# Autodesk Inventor assembly: Stand
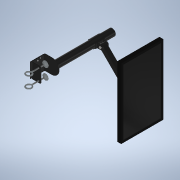
[picture p0: Inventor's stored thumbnail of the model, 180x180]
Saved by Autodesk Inventor 2020 (Build 240168000, 168)
## iProperties
Created: 2021-07-08
Part Number: Stand
Document SubType Name: Assembly
Designer: Simon.Alvarez
Mass: 3004.31 g
Surface Area: 3337 cm^2
Volume: 382.876 cm^3
Density: 7.84669 g/cm^3
Author: Simon.Alvarez
## Documents named in this file (9)
- C:\Users\Simon.Alvarez\Desktop\Simon off laptop\Desk\Monitor Stand\Stand.iam
- C:\Users\Simon.Alvarez\Desktop\Simon off laptop\Desk\Monitor Stand\Pole.ipt
- C:\Users\Simon.Alvarez\Desktop\Simon off laptop\Desk\Monitor Stand\Clamp_Plate.ipt
- C:\Users\Simon.Alvarez\Documents\Inventor\Content Center Files\R2020\en-US\BS EN ISO 7045 Z\EN ISO 7045 - M8 x 10 - 4.8 - Z(1).ipt
- C:\Users\Simon.Alvarez\Desktop\Simon off laptop\Desk\Monitor Stand\Clamp Thread.ipt
- C:\Users\Simon.Alvarez\Documents\Inventor\Content Center Files\R2020\en-US\BS EN ISO 7045 Z\EN ISO 7045 - M6 x 12 - 4.8 - Z(1).ipt
- C:\Users\Simon.Alvarez\Desktop\Simon off laptop\Desk\Monitor Stand\Arm.iam
- C:\Users\Simon.Alvarez\Desktop\Simon off laptop\Desk\Monitor Stand\Monitor_21inch.ipt
- C:\Users\Simon.Alvarez\Documents\Inventor\Content Center Files\R2020\en-US\BS EN ISO 7045 Z\EN ISO 7045 - M4 x 5 - 4.8 - Z(1).ipt
## Components (14 placed, 8 different names)
1. Pole:1 — Flush:1, Flush:2, Flush:3, Mate:1, Mate:2, Mate:3, Insert:1, Insert:2, Mate:7, Mate:8
2. Clamp_Plate:1 — Mate:1, Mate:2, Mate:3, Mate:4, Mate:5
3. BS EN ISO 7045 Z - Metric M8 x 10 - 4.8 - Z:1 — Insert:1
4. BS EN ISO 7045 Z - Metric M8 x 10 - 4.8 - Z:2 — Insert:2
5. Clamp Thread:1 — Mate:4, Mate:6
6. Clamp Thread:2 — Mate:5, Mate:6
7. Arm:1 [sub-assembly] — Mate:7, Mate:8, Mate:9, Tangent:1, Mate:10, Tangent:2, Mate:11, Mate:12, Mate:13, Insert:3, Insert:4, Insert:5, Insert:6
8. BS EN ISO 7045 Z - Metric M6 x 12 - 4.8 - Z:1 — Mate:9, Tangent:1
9. BS EN ISO 7045 Z - Metric M6 x 12 - 4.8 - Z:2 — Mate:10, Tangent:2
10. Monitor_21inch:1 — Mate:11, Mate:12, Mate:13
11. BS EN ISO 7045 Z - Metric M4 x 5 - 4.8 - Z:1 — Insert:3
12. BS EN ISO 7045 Z - Metric M4 x 5 - 4.8 - Z:2 — Insert:4
13. BS EN ISO 7045 Z - Metric M4 x 5 - 4.8 - Z:3 — Insert:5
14. BS EN ISO 7045 Z - Metric M4 x 5 - 4.8 - Z:4 — Insert:6
## Relationships (24: Mate 13, Insert 6, Flush 3, Tangent 2)
- Flush:1: Pole:1
- Flush:2: Pole:1
- Flush:3: Pole:1
- Mate:1: Pole:1 ↔ Clamp_Plate:1
- Mate:2: Pole:1 ↔ Clamp_Plate:1
- Mate:3: Pole:1 ↔ Clamp_Plate:1
- Insert:1: Pole:1 ↔ BS EN ISO 7045 Z - Metric M8 x 10 - 4.8 - Z:1
- Insert:2: Pole:1 ↔ BS EN ISO 7045 Z - Metric M8 x 10 - 4.8 - Z:2
- Mate:4: Clamp_Plate:1 ↔ Clamp Thread:1
- Mate:5: Clamp_Plate:1 ↔ Clamp Thread:2
- Mate:6: Clamp Thread:1 ↔ Clamp Thread:2
- Mate:7: Pole:1 ↔ Arm:1
- Mate:8: Pole:1 ↔ Arm:1
- Mate:9: Arm:1 ↔ BS EN ISO 7045 Z - Metric M6 x 12 - 4.8 - Z:1
- Tangent:1: Arm:1 ↔ BS EN ISO 7045 Z - Metric M6 x 12 - 4.8 - Z:1
- Mate:10: Arm:1 ↔ BS EN ISO 7045 Z - Metric M6 x 12 - 4.8 - Z:2
- Tangent:2: Arm:1 ↔ BS EN ISO 7045 Z - Metric M6 x 12 - 4.8 - Z:2
- Mate:11: Arm:1 ↔ Monitor_21inch:1
- Mate:12: Arm:1 ↔ Monitor_21inch:1
- Mate:13: Arm:1 ↔ Monitor_21inch:1
- Insert:3: Arm:1 ↔ BS EN ISO 7045 Z - Metric M4 x 5 - 4.8 - Z:1
- Insert:4: Arm:1 ↔ BS EN ISO 7045 Z - Metric M4 x 5 - 4.8 - Z:2
- Insert:5: Arm:1 ↔ BS EN ISO 7045 Z - Metric M4 x 5 - 4.8 - Z:3
- Insert:6: Arm:1 ↔ BS EN ISO 7045 Z - Metric M4 x 5 - 4.8 - Z:4
